# Autodesk Inventor assembly: GE-20020_Vinyl Blue_Axle
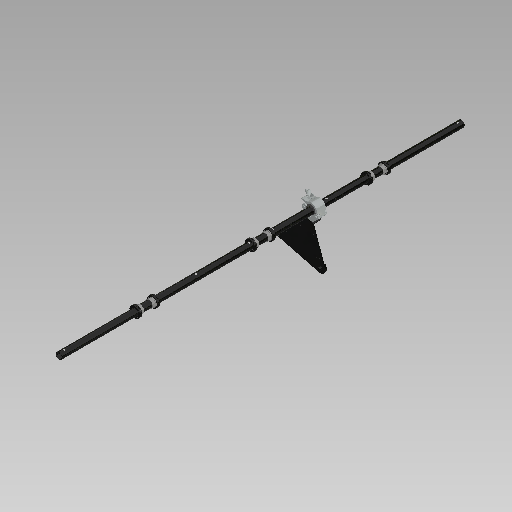
[picture p0: Inventor's stored thumbnail of the model, 512x512]
Saved by Autodesk Inventor 2020.1 (Build 241239000, 239)
## iProperties
Created: 2019-10-14
Part Number: GE-20020_Vinyl Blue_Axle
Document SubType Name: Assembly
Designer: Phillips Lenovo
Author: Phillips Lenovo
Revision Number: ANY
## Documents named in this file (12)
- D:\FIRST 2020\FRC 2020\FRC Field 2020\Parts\GE-20020_Vinyl Blue_Axle.iam
- D:\FIRST 2020\FRC 2020\FRC Field 2020\Parts\pin_clevis_.25_1.75_pin_clevis_.25_1.75.ipt
- D:\FIRST 2020\FRC 2020\FRC Field 2020\Parts\pin_cotter_.0625_.50_pin_cotter_.0625_.50.ipt
- D:\FIRST 2020\FRC 2020\FRC Field 2020\Parts\hex_.5_20_1.75_92865A732.ipt
- D:\FIRST 2020\FRC 2020\FRC Field 2020\Parts\washer_flat_.5_98023A029.ipt
- D:\FIRST 2020\FRC 2020\FRC Field 2020\Parts\nylock_.50_20_95615A220.ipt
- D:\FIRST 2020\FRC 2020\FRC Field 2020\Parts\GE-20015.ipt
- D:\FIRST 2020\FRC 2020\FRC Field 2020\Parts\6435K230_ONE-PIECE CLAMP-ON SHAFT COLLAR_6435K23.ipt
- D:\FIRST 2020\FRC 2020\FRC Field 2020\Parts\GE-20013.ipt
- D:\FIRST 2020\FRC 2020\FRC Field 2020\Parts\3126T310_RAILING CLAMP_KC_3126T31.ipt
- D:\FIRST 2020\FRC 2020\FRC Field 2020\Parts\hanger sensor.ipt
- D:\FIRST 2020\FRC 2020\FRC Field 2020\Parts\GE-20014.ipt
## Components (32 placed, 32 different names)
1. pin_clevis_.25_1.75_pin_clevis_.25_1.75_519
2. pin_cotter_.0625_.50_pin_cotter_.0625_.50_520
3. hex_.5_20_1.75_92865A732_521
4. washer_flat_.5_98023A029_522
5. nylock_.50_20_95615A220_523
6. GE-20015_540
7. GE-20015_541
8. GE-20015_542
9. GE-20015_543
10. GE-20015_544
11. GE-20015_545
12. 6435K230_ONE-PIECE CLAMP-ON SHAFT COLLAR_6435K23_546
13. 6435K230_ONE-PIECE CLAMP-ON SHAFT COLLAR_6435K23_547
14. 6435K230_ONE-PIECE CLAMP-ON SHAFT COLLAR_6435K23_548 — Insert:5
15. 6435K230_ONE-PIECE CLAMP-ON SHAFT COLLAR_6435K23_549 — Insert:4, Insert:5
16. 6435K230_ONE-PIECE CLAMP-ON SHAFT COLLAR_6435K23_550
17. 6435K230_ONE-PIECE CLAMP-ON SHAFT COLLAR_6435K23_551
18. GE-20013_552 — Insert:4
19. pin_cotter_.0625_.50_pin_cotter_.0625_.50_586
20. pin_clevis_.25_1.75_pin_clevis_.25_1.75_587
21. pin_cotter_.0625_.50_pin_cotter_.0625_.50_588
22. pin_cotter_.0625_.50_pin_cotter_.0625_.50_589
23. pin_clevis_.25_1.75_pin_clevis_.25_1.75_590
24. pin_clevis_.25_1.75_pin_clevis_.25_1.75_591
25. 3126T310_RAILING CLAMP_KC_3126T31_592
26. hanger sensor_593
27. hanger sensor_594
28. GE-20014_595
29. pin_cotter_.0625_.50_pin_cotter_.0625_.50_596
30. pin_cotter_.0625_.50_pin_cotter_.0625_.50_597
31. pin_clevis_.25_1.75_pin_clevis_.25_1.75_598
32. pin_clevis_.25_1.75_pin_clevis_.25_1.75_599
## Relationships (2: Insert 2)
- Insert:4 (430.0982 mm): 6435K230_ONE-PIECE CLAMP-ON SHAFT COLLAR_6435K23_549 ↔ GE-20013_552
- Insert:5 (-114.3 mm): 6435K230_ONE-PIECE CLAMP-ON SHAFT COLLAR_6435K23_548 ↔ 6435K230_ONE-PIECE CLAMP-ON SHAFT COLLAR_6435K23_549
